# Autodesk Inventor assembly: main_assembly
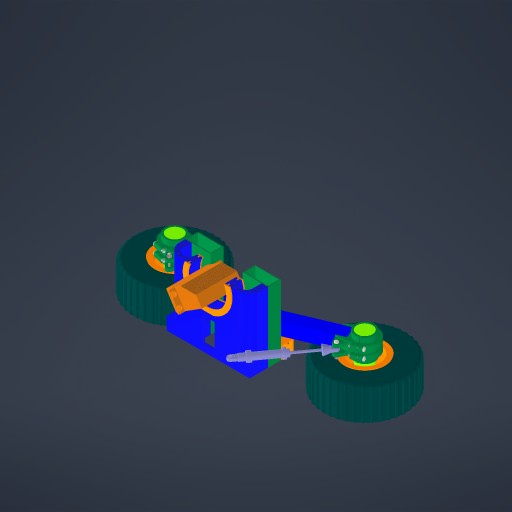
[picture p0: Inventor's stored thumbnail of the model, 512x512]
Saved by Autodesk Inventor 2024 (Build 280153000, 153)
## iProperties
Created: 2023-09-26
Part Number: main_assembly
Document SubType Name: Assembly
Designer: user
Author: user
## Documents named in this file (9)
- D:\Docs\Robot\3d_v2\main_assembly.iam
- D:\Docs\Robot\3d_v2\base\base_assambly.iam
- D:\Docs\Robot\3d_v2\machine_body\arm_assembly_r.iam
- D:\Docs\Robot\3d_v2\machine_body\arm_assembly_l.iam
- D:\Docs\Robot\3d_v2\default_components\shock_absorber.ipt
- D:\Docs\Robot\3d_v2\electronics\Battery_18650_asembly.iam
- D:\Docs\Robot\3d_v2\electronics\Arduino MEGA 2560 R3.ipt
- D:\Docs\Robot\3d_v2\electronics\BTS7960\BTS7960.iam
- D:\Docs\Robot\3d_v2\machine_body\manipulator.iam
## Components (11 placed, 8 different names)
1. base_assambly:1 [sub-assembly] — Совмещение:1, Совмещение:2, Совмещение:3, Вставка:8, Вставка:9, Вставка:10, Вставка:11, Заподлицо:1, Совмещение:4, Заподлицо:2
2. arm_assembly_r:1 [sub-assembly] — Вставка:11
3. arm_assembly_l:1 [sub-assembly] — Вставка:8
4. shock_absorber:1 — Вставка:12
5. arm_assembly_l:2 [sub-assembly] — Вставка:9, Вставка:12
6. arm_assembly_r:2 [sub-assembly] — Вставка:10
7. Battery_18650_asembly:1 [sub-assembly]
8. Arduino MEGA 2560 R3:1
9. BTS7960:1 [sub-assembly]
10. BTS7960:2 [sub-assembly]
11. manipulator:1 [sub-assembly] — Заподлицо:1, Совмещение:4, Заподлицо:2
## Relationships (11: Insert 5, Mate 4, Flush 2)
- Совмещение:1 [Mate]: base_assambly:1
- Совмещение:2 [Mate]: base_assambly:1
- Совмещение:3 [Mate]: base_assambly:1
- Вставка:8 [Insert]: base_assambly:1 ↔ arm_assembly_l:1
- Вставка:9 [Insert]: base_assambly:1 ↔ arm_assembly_l:2
- Вставка:10 [Insert]: base_assambly:1 ↔ arm_assembly_r:2
- Вставка:11 [Insert]: base_assambly:1 ↔ arm_assembly_r:1
- Вставка:12 [Insert]: shock_absorber:1 ↔ arm_assembly_l:2
- Заподлицо:1 [Flush]: base_assambly:1 ↔ manipulator:1
- Совмещение:4 [Mate]: base_assambly:1 ↔ manipulator:1
- Заподлицо:2 [Flush]: base_assambly:1 ↔ manipulator:1
